# Autodesk Inventor assembly: body
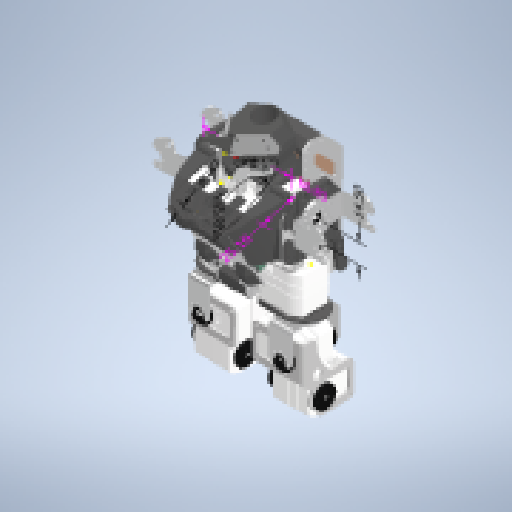
[picture p0: Inventor's stored thumbnail of the model, 512x512]
Saved by Autodesk Inventor 2024.1 (Build 281209000, 209)
## iProperties
Created: 2024-10-10
Part Number: body
Document SubType Name: Assembly
Designer: hibik
Author: hibik
## Documents named in this file (6)
- C:\Users\hibik\Documents\Robomech\HR\Eglantyne\hard\body.iam
- C:\Users\hibik\Documents\Robomech\HR\Eglantyne\hard\under_body\under_body.iam
- C:\Users\hibik\Documents\Robomech\HR\Eglantyne\hard\upper_body\upperbody.iam
- C:\Users\hibik\Documents\Robomech\HR\Eglantyne\hard\needed_model\battely.ipt
- C:\Users\hibik\Documents\Robomech\HR\Eglantyne\hard\head\head.iam
- C:\Users\hibik\Documents\Robomech\HR\Eglantyne\hard\arm\sholder.ipt
## Components (5 placed, 5 different names)
1. under_body:1 [sub-assembly] — フラッシュ:1, メイト:1, フラッシュ:2
2. battely:1
3. upperbody:1 [sub-assembly] — フラッシュ:1, メイト:1, フラッシュ:2, 挿入:1, 挿入:2, 挿入:3
4. head:1 [sub-assembly] — 挿入:1, 挿入:2
5. sholder:1 — 挿入:3
## Relationships (6: Insert 3, Flush 2, Mate 1)
- フラッシュ:1 [Flush]: under_body:1 ↔ upperbody:1
- メイト:1 [Mate]: under_body:1 ↔ upperbody:1
- フラッシュ:2 [Flush]: under_body:1 ↔ upperbody:1
- 挿入:1 [Insert]: upperbody:1 ↔ head:1
- 挿入:2 [Insert]: upperbody:1 ↔ head:1
- 挿入:3 [Insert] (0.2 mm): upperbody:1 ↔ sholder:1
